# Autodesk Inventor assembly: カート
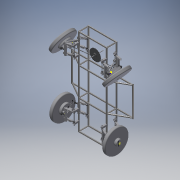
[picture p0: Inventor's stored thumbnail of the model, 180x180]
Saved by Autodesk Inventor 2018 (Build 220112000, 112)
## iProperties
Created: 2017-10-07
Part Number: カート
Material: 一般
Document SubType Name: Assembly
Designer: Kosei
Author: Kosei
## Documents named in this file (26)
- D:\Works\RBBR\CAD\カート.iam
- D:\Works\RBBR\CAD\シャーシ\シャーシ.iam
- D:\Works\RBBR\CAD\サスペンション\上アーム(前).iam
- D:\Works\RBBR\CAD\汎用部品\シャフト12x300mm.ipt
- D:\Works\RBBR\CAD\サスペンション\下アーム(前後).iam
- D:\Works\RBBR\CAD\サスペンション\車軸受け(前,左).iam
- D:\Works\RBBR\CAD\汎用部品\シャフト10x230mm.ipt
- D:\Works\RBBR\CAD\サスペンション\スプリング\スプリング.iam
- D:\Works\RBBR\CAD\車輪\前輪.ipt
- D:\Works\RBBR\CAD\車輪\前輪シャフト.ipt
- D:\Works\RBBR\CAD\車輪\前輪シャフトワッシャー.ipt
- D:\Works\RBBR\CAD\サスペンション\車軸受け(前,右).iam
- D:\Works\RBBR\CAD\ステアリング\ロッド.iam
- D:\Works\RBBR\CAD\ステアリング\車輪側スプロケット.ipt
- D:\Works\RBBR\CAD\装飾(仮)\前後.ipt
- D:\Works\RBBR\CAD\装飾(仮)\左右.ipt
- D:\Works\RBBR\CAD\装飾(仮)\泥除け1.ipt
- D:\Works\RBBR\CAD\装飾(仮)\床板.ipt
- D:\Works\RBBR\CAD\装飾(仮)\泥除け2.ipt
- D:\Works\RBBR\CAD\装飾(仮)\泥除け3.ipt
- D:\Works\RBBR\CAD\装飾(仮)\泥除け4.ipt
- D:\Works\RBBR\CAD\サスペンション\上アーム(後).iam
- D:\Works\RBBR\CAD\サスペンション\車軸受け(後,右).iam
- D:\Works\RBBR\CAD\車輪\後輪.ipt
- D:\Works\RBBR\CAD\車輪\後輪シャフト.ipt
- D:\Works\RBBR\CAD\サスペンション\車軸受け(後,左).iam
## Components (55 placed, 25 different names)
1. シャーシ:1 [sub-assembly] — フラッシュ:2, フラッシュ:3, フラッシュ:4, 円柱状:1, フラッシュ:5, 円柱状:2, フラッシュ:6, 円柱状:3, フラッシュ:7, 円柱状:4, フラッシュ:8, メイト:1, メイト:2, メイト:3, メイト:4, フラッシュ:9, フラッシュ:10, メイト:5, フラッシュ:11, メイト:6, フラッシュ:12, 角度:3, メイト:7, フラッシュ:13, フラッシュ:14, メイト:8, フラッシュ:15, フラッシュ:16, メイト:9, フラッシュ:17, フラッシュ:18, メイト:10, フラッシュ:19, メイト:12, フラッシュ:25, メイト:15, メイト:21, メイト:24, メイト:25, メイト:27, 円柱状:16, フラッシュ:29, 円柱状:17, フラッシュ:30, メイト:41, メイト:42, フラッシュ:31, 角度:9, 円柱状:22, フラッシュ:32, 円柱状:23, フラッシュ:33, メイト:43, メイト:44, 角度:10
2. シャフト12x300mm:1 — 円柱状:1, フラッシュ:5, 円柱状:5, 円柱状:11
3. シャフト12x300mm:3 — 円柱状:3, フラッシュ:7, 円柱状:7
4. シャフト10x230mm:1 — 円柱状:9, フラッシュ:9, 円柱状:12
5. 上アーム(前):1 [sub-assembly] — 円柱状:5, メイト:1, リジッド:1, 角度:11
6. 下アーム(前後):1 [sub-assembly] — 円柱状:7, メイト:3, リジッド:2, 円柱状:9
7. 車軸受け(前,左):1 [sub-assembly] — リジッド:1, リジッド:2, 回転:2, リジッド:9
8. スプリング:1 [sub-assembly] — 円柱状:11, 円柱状:12
9. 前輪:1 — 回転:1, リジッド:5
10. 前輪シャフト:1 — 回転:1
11. 前輪シャフトワッシャー:1 — リジッド:5, 回転:2
12. シャフト12x300mm:2 — 円柱状:2, フラッシュ:6, 円柱状:6, 円柱状:13
13. シャフト12x300mm:4 — 円柱状:4, フラッシュ:8, 円柱状:8
14. シャフト10x230mm:2 — フラッシュ:10, 円柱状:10, 円柱状:14
15. 上アーム(前):2 [sub-assembly] — 円柱状:6, メイト:2, リジッド:3, 角度:5
16. 下アーム(前後):2 [sub-assembly] — 円柱状:8, メイト:4, リジッド:4, 円柱状:10
17. 車軸受け(前,右):1 [sub-assembly] — リジッド:3, リジッド:4, 回転:3, リジッド:8
18. スプリング:2 [sub-assembly] — 円柱状:13, 円柱状:14
19. 前輪:2 — リジッド:6, リジッド:7
20. 前輪シャフト:2 — リジッド:6
21. 前輪シャフトワッシャー:2 — リジッド:7, 回転:3
22. シャフト12x300mm:6 — 円柱状:16, フラッシュ:29, 円柱状:18, 円柱状:21
23. シャフト12x300mm:7 — 円柱状:17, フラッシュ:30, 円柱状:19
24. 上アーム(後):1 [sub-assembly] — 円柱状:18, メイト:41, リジッド:14, リジッド:15, 円柱状:21
25. 下アーム(前後):3 [sub-assembly] — 円柱状:19, メイト:42, 円柱状:20, リジッド:16
26. シャフト10x230mm:3 — 円柱状:20, フラッシュ:31
27. 車軸受け(後,右):1 [sub-assembly] — リジッド:14, リジッド:15, リジッド:16, 回転:4
28. 後輪:1 — 回転:23, 回転:4, 角度:9
29. 後輪シャフト:1 — 回転:23
30. シャフト12x300mm:8 — 円柱状:22, フラッシュ:32, 円柱状:24, 円柱状:25
31. シャフト12x300mm:9 — 円柱状:23, フラッシュ:33, 円柱状:26, 円柱状:27
32. 上アーム(後):2 [sub-assembly] — 円柱状:24, 円柱状:25, メイト:43, リジッド:19, リジッド:20
33. 車軸受け(後,左):1 [sub-assembly] — リジッド:18, リジッド:19, リジッド:20, 回転:22
34. 下アーム(前後):4 [sub-assembly] — 円柱状:26, 円柱状:27, メイト:44, リジッド:18
35. 後輪:2 — 回転:5, 回転:22, 角度:10
36. 後輪シャフト:2 — 回転:5
37. ロッド:1 [sub-assembly] — リジッド:8, リジッド:12, 角度:6
38. ロッド:2 [sub-assembly] — リジッド:9, リジッド:13, 角度:7
39. 車輪側スプロケット:1 — 円柱状:15, フラッシュ:12, リジッド:12, リジッド:13, 角度:3, 角度:6, 角度:7
40. シャフト12x300mm:5 — メイト:5, フラッシュ:11, メイト:6, 円柱状:15
41. 前後:1 — メイト:7, フラッシュ:13, フラッシュ:14, メイト:19, メイト:36, メイト:37
42. 前後:2 — メイト:8, フラッシュ:15, フラッシュ:16, メイト:22
43. 左右:1 — メイト:9, フラッシュ:17, フラッシュ:18, フラッシュ:26, メイト:16, フラッシュ:27, フラッシュ:28, メイト:26
44. 左右:2 — メイト:10, フラッシュ:19, フラッシュ:23, フラッシュ:24, フラッシュ:25, メイト:14, メイト:20, メイト:23, メイト:28
45. 泥除け1:1 — メイト:27, フラッシュ:24, メイト:28, メイト:35
46. 泥除け1:2 — メイト:15, フラッシュ:26, メイト:16, メイト:34
47. 泥除け1:3 — メイト:12, フラッシュ:23, メイト:14
48. 泥除け1:4 — フラッシュ:27, メイト:25, フラッシュ:28, メイト:26
49. 泥除け2:1 — メイト:30, メイト:35, メイト:36, メイト:38, メイト:39, メイト:40
50. 泥除け2:2 — メイト:33, メイト:34, メイト:37
51. 泥除け3:1 — メイト:38
52. 泥除け3:2 — メイト:39
53. 泥除け4:1 — メイト:40
54. 床板:1 — メイト:22, メイト:23, メイト:24
55. 床板:2 — メイト:19, メイト:20, メイト:21, メイト:30, メイト:33
## Relationships (124: Mate 37, Flush 29, CylindricalJoint 27, WeldJoint 17, RevoluteJoint 7, Angle 7)
- フラッシュ:2 [Flush]: シャーシ:1
- フラッシュ:3 [Flush]: シャーシ:1
- フラッシュ:4 [Flush]: シャーシ:1
- 円柱状:1 [CylindricalJoint]: シャーシ:1 ↔ シャフト12x300mm:1
- フラッシュ:5 [Flush]: シャーシ:1 ↔ シャフト12x300mm:1
- 円柱状:2 [CylindricalJoint]: シャーシ:1 ↔ シャフト12x300mm:2
- フラッシュ:6 [Flush]: シャーシ:1 ↔ シャフト12x300mm:2
- 円柱状:3 [CylindricalJoint]: シャーシ:1 ↔ シャフト12x300mm:3
- フラッシュ:7 [Flush]: シャーシ:1 ↔ シャフト12x300mm:3
- 円柱状:4 [CylindricalJoint]: シャーシ:1 ↔ シャフト12x300mm:4
- フラッシュ:8 [Flush]: シャーシ:1 ↔ シャフト12x300mm:4
- 円柱状:5 [CylindricalJoint]: シャフト12x300mm:1 ↔ 上アーム(前):1
- メイト:1 [Mate]: シャーシ:1 ↔ 上アーム(前):1
- 円柱状:6 [CylindricalJoint]: シャフト12x300mm:2 ↔ 上アーム(前):2
- メイト:2 [Mate]: シャーシ:1 ↔ 上アーム(前):2
- 円柱状:7 [CylindricalJoint]: シャフト12x300mm:3 ↔ 下アーム(前後):1
- メイト:3 [Mate]: シャーシ:1 ↔ 下アーム(前後):1
- 円柱状:8 [CylindricalJoint]: シャフト12x300mm:4 ↔ 下アーム(前後):2
- メイト:4 [Mate]: シャーシ:1 ↔ 下アーム(前後):2
- リジッド:1 [WeldJoint]: 上アーム(前):1 ↔ 車軸受け(前,左):1
- リジッド:2 [WeldJoint]: 下アーム(前後):1 ↔ 車軸受け(前,左):1
- リジッド:3 [WeldJoint]: 上アーム(前):2 ↔ 車軸受け(前,右):1
- リジッド:4 [WeldJoint]: 下アーム(前後):2 ↔ 車軸受け(前,右):1
- 円柱状:9 [CylindricalJoint]: シャフト10x230mm:1 ↔ 下アーム(前後):1
- フラッシュ:9 [Flush]: シャーシ:1 ↔ シャフト10x230mm:1
- フラッシュ:10 [Flush]: シャーシ:1 ↔ シャフト10x230mm:2
- 円柱状:10 [CylindricalJoint]: シャフト10x230mm:2 ↔ 下アーム(前後):2
- 円柱状:11 [CylindricalJoint]: シャフト12x300mm:1 ↔ スプリング:1
- 円柱状:12 [CylindricalJoint]: シャフト10x230mm:1 ↔ スプリング:1
- 円柱状:13 [CylindricalJoint]: シャフト12x300mm:2 ↔ スプリング:2
- 円柱状:14 [CylindricalJoint]: シャフト10x230mm:2 ↔ スプリング:2
- 回転:1 [RevoluteJoint]: 前輪:1 ↔ 前輪シャフト:1
- リジッド:5 [WeldJoint]: 前輪:1 ↔ 前輪シャフトワッシャー:1
- 回転:2 [RevoluteJoint]: 車軸受け(前,左):1 ↔ 前輪シャフトワッシャー:1
- リジッド:6 [WeldJoint]: 前輪:2 ↔ 前輪シャフト:2
- リジッド:7 [WeldJoint]: 前輪:2 ↔ 前輪シャフトワッシャー:2
- 回転:3 [RevoluteJoint]: 車軸受け(前,右):1 ↔ 前輪シャフトワッシャー:2
- リジッド:8 [WeldJoint]: 車軸受け(前,右):1 ↔ ロッド:1
- リジッド:9 [WeldJoint]: 車軸受け(前,左):1 ↔ ロッド:2
- メイト:5 [Mate]: シャーシ:1 ↔ シャフト12x300mm:5
- フラッシュ:11 [Flush]: シャーシ:1 ↔ シャフト12x300mm:5
- メイト:6 [Mate]: シャーシ:1 ↔ シャフト12x300mm:5
- 円柱状:15 [CylindricalJoint]: 車輪側スプロケット:1 ↔ シャフト12x300mm:5
- フラッシュ:12 [Flush] (160 mm): シャーシ:1 ↔ 車輪側スプロケット:1
- リジッド:12 [WeldJoint]: ロッド:1 ↔ 車輪側スプロケット:1
- リジッド:13 [WeldJoint]: ロッド:2 ↔ 車輪側スプロケット:1
- 角度:3 [Angle] (10 deg): シャーシ:1 ↔ 車輪側スプロケット:1
- 角度:5 [Angle] (10 deg): 上アーム(前):2
- 角度:6 [Angle] (0 deg): ロッド:1 ↔ 車輪側スプロケット:1
- 角度:7 [Angle] (0 deg): ロッド:2 ↔ 車輪側スプロケット:1
- メイト:7 [Mate]: シャーシ:1 ↔ 前後:1
- フラッシュ:13 [Flush] (40 mm): シャーシ:1 ↔ 前後:1
- フラッシュ:14 [Flush] (640 mm): シャーシ:1 ↔ 前後:1
- メイト:8 [Mate]: シャーシ:1 ↔ 前後:2
- フラッシュ:15 [Flush] (40 mm): シャーシ:1 ↔ 前後:2
- フラッシュ:16 [Flush] (640 mm): シャーシ:1 ↔ 前後:2
- メイト:9 [Mate]: シャーシ:1 ↔ 左右:1
- フラッシュ:17 [Flush] (40 mm): シャーシ:1 ↔ 左右:1
- フラッシュ:18 [Flush] (4 mm): シャーシ:1 ↔ 左右:1
- メイト:10 [Mate]: シャーシ:1 ↔ 左右:2
- フラッシュ:19 [Flush] (40 mm): シャーシ:1 ↔ 左右:2
- メイト:12 [Mate]: シャーシ:1 ↔ 泥除け1:3
- フラッシュ:23 [Flush]: 左右:2 ↔ 泥除け1:3
- メイト:27 [Mate]: シャーシ:1 ↔ 泥除け1:1
- フラッシュ:24 [Flush]: 左右:2 ↔ 泥除け1:1
- フラッシュ:25 [Flush] (4 mm): シャーシ:1 ↔ 左右:2
- メイト:14 [Mate]: 左右:2 ↔ 泥除け1:3
- メイト:15 [Mate]: シャーシ:1 ↔ 泥除け1:2
- フラッシュ:26 [Flush]: 左右:1 ↔ 泥除け1:2
- メイト:16 [Mate]: 左右:1 ↔ 泥除け1:2
- フラッシュ:27 [Flush]: 左右:1 ↔ 泥除け1:4
- メイト:19 [Mate]: 前後:1 ↔ 床板:2
- メイト:20 [Mate]: 左右:2 ↔ 床板:2
- メイト:21 [Mate]: シャーシ:1 ↔ 床板:2
- メイト:22 [Mate]: 前後:2 ↔ 床板:1
- メイト:23 [Mate]: 左右:2 ↔ 床板:1
- メイト:24 [Mate]: シャーシ:1 ↔ 床板:1
- メイト:25 [Mate]: シャーシ:1 ↔ 泥除け1:4
- フラッシュ:28 [Flush]: 左右:1 ↔ 泥除け1:4
- メイト:26 [Mate]: 左右:1 ↔ 泥除け1:4
- メイト:28 [Mate]: 左右:2 ↔ 泥除け1:1
- メイト:30 [Mate]: 泥除け2:1 ↔ 床板:2
- メイト:33 [Mate]: 泥除け2:2 ↔ 床板:2
- メイト:34 [Mate]: 泥除け1:2 ↔ 泥除け2:2
- メイト:35 [Mate]: 泥除け1:1 ↔ 泥除け2:1
- メイト:36 [Mate]: 前後:1 ↔ 泥除け2:1
- メイト:37 [Mate]: 前後:1 ↔ 泥除け2:2
- メイト:38 [Mate]: 泥除け2:1 ↔ 泥除け3:1
- メイト:39 [Mate]: 泥除け2:1 ↔ 泥除け3:2
- メイト:40 [Mate]: 泥除け2:1 ↔ 泥除け4:1
- 円柱状:16 [CylindricalJoint]: シャーシ:1 ↔ シャフト12x300mm:6
- フラッシュ:29 [Flush]: シャーシ:1 ↔ シャフト12x300mm:6
- 円柱状:17 [CylindricalJoint]: シャーシ:1 ↔ シャフト12x300mm:7
- フラッシュ:30 [Flush]: シャーシ:1 ↔ シャフト12x300mm:7
- 円柱状:18 [CylindricalJoint]: シャフト12x300mm:6 ↔ 上アーム(後):1
- メイト:41 [Mate]: シャーシ:1 ↔ 上アーム(後):1
- 円柱状:19 [CylindricalJoint]: シャフト12x300mm:7 ↔ 下アーム(前後):3
- メイト:42 [Mate]: シャーシ:1 ↔ 下アーム(前後):3
- 円柱状:20 [CylindricalJoint]: 下アーム(前後):3 ↔ シャフト10x230mm:3
- フラッシュ:31 [Flush]: シャーシ:1 ↔ シャフト10x230mm:3
- リジッド:14 [WeldJoint]: 上アーム(後):1 ↔ 車軸受け(後,右):1
- リジッド:15 [WeldJoint]: 上アーム(後):1 ↔ 車軸受け(後,右):1
- 円柱状:21 [CylindricalJoint]: シャフト12x300mm:6 ↔ 上アーム(後):1
- リジッド:16 [WeldJoint]: 下アーム(前後):3 ↔ 車軸受け(後,右):1
- 回転:23 [RevoluteJoint]: 後輪:1 ↔ 後輪シャフト:1
- 回転:4 [RevoluteJoint]: 車軸受け(後,右):1 ↔ 後輪:1
- 角度:9 [Angle] (180 deg): シャーシ:1 ↔ 後輪:1
- 円柱状:22 [CylindricalJoint]: シャーシ:1 ↔ シャフト12x300mm:8
- フラッシュ:32 [Flush]: シャーシ:1 ↔ シャフト12x300mm:8
- 円柱状:23 [CylindricalJoint]: シャーシ:1 ↔ シャフト12x300mm:9
- フラッシュ:33 [Flush]: シャーシ:1 ↔ シャフト12x300mm:9
- 円柱状:24 [CylindricalJoint]: シャフト12x300mm:8 ↔ 上アーム(後):2
- 円柱状:25 [CylindricalJoint]: シャフト12x300mm:8 ↔ 上アーム(後):2
- メイト:43 [Mate]: シャーシ:1 ↔ 上アーム(後):2
- 円柱状:26 [CylindricalJoint]: シャフト12x300mm:9 ↔ 下アーム(前後):4
- 円柱状:27 [CylindricalJoint]: シャフト12x300mm:9 ↔ 下アーム(前後):4
- メイト:44 [Mate]: シャーシ:1 ↔ 下アーム(前後):4
- リジッド:18 [WeldJoint]: 車軸受け(後,左):1 ↔ 下アーム(前後):4
- リジッド:19 [WeldJoint]: 上アーム(後):2 ↔ 車軸受け(後,左):1
- リジッド:20 [WeldJoint]: 上アーム(後):2 ↔ 車軸受け(後,左):1
- 回転:5 [RevoluteJoint]: 後輪:2 ↔ 後輪シャフト:2
- 回転:22 [RevoluteJoint]: 車軸受け(後,左):1 ↔ 後輪:2
- 角度:10 [Angle] (0 deg): シャーシ:1 ↔ 後輪:2
- 角度:11 [Angle] (15 deg): 上アーム(前):1
